# Autodesk Inventor assembly: SingleOmniWheelAssembly
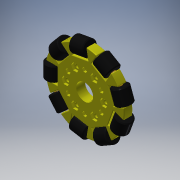
[picture p0: Inventor's stored thumbnail of the model, 180x180]
Saved by Autodesk Inventor 2016 (Build 200138000, 138)
## iProperties
Created: 2016-12-01
Part Number: SingleOmniWheelAssembly
Document SubType Name: Assembly
Designer: Evan Phil George
Author: Evan Phil George
## Documents named in this file (3)
- C:\Users\Evan Phil George\Desktop\Ball Balancing Robot\TestBenchInventor\OmniWheel\SingleOmniWheelAssembly.iam
- C:\Users\Evan Phil George\Desktop\Ball Balancing Robot\TestBenchInventor\OmniWheel\Frame.ipt
- C:\Users\Evan Phil George\Desktop\Ball Balancing Robot\TestBenchInventor\OmniWheel\RollerAxleWasherSubAssembly.iam
## Components (11 placed, 2 different names)
1. Frame:1 — Mate:1, Mate:2, Mate:3, Mate:4, Mate:5, Mate:6, Mate:7, Mate:8, Mate:9, Mate:10, Mate:11, Mate:12, Mate:13, Mate:14, Mate:15, Mate:16, Mate:17, Mate:18, Mate:19, Mate:20, Mate:21
2. RollerAxleWasherSubAssembly:1 [sub-assembly] — Mate:1, Mate:2
3. RollerAxleWasherSubAssembly:2 [sub-assembly] — Mate:3, Mate:4
4. RollerAxleWasherSubAssembly:3 [sub-assembly] — Mate:5, Mate:6
5. RollerAxleWasherSubAssembly:4 [sub-assembly] — Mate:7, Mate:8
6. RollerAxleWasherSubAssembly:5 [sub-assembly] — Mate:9, Mate:10
7. RollerAxleWasherSubAssembly:6 [sub-assembly] — Mate:11, Mate:12
8. RollerAxleWasherSubAssembly:7 [sub-assembly] — Mate:13, Mate:14
9. RollerAxleWasherSubAssembly:8 [sub-assembly] — Mate:15, Mate:16
10. RollerAxleWasherSubAssembly:9 [sub-assembly] — Mate:17, Mate:18
11. Frame:2 — Mate:19, Mate:20, Mate:21
## Relationships (21: Mate 21)
- Mate:1: Frame:1 ↔ RollerAxleWasherSubAssembly:1
- Mate:2 (0.5 mm): Frame:1 ↔ RollerAxleWasherSubAssembly:1
- Mate:3: Frame:1 ↔ RollerAxleWasherSubAssembly:2
- Mate:4 (0.5 mm): Frame:1 ↔ RollerAxleWasherSubAssembly:2
- Mate:5: Frame:1 ↔ RollerAxleWasherSubAssembly:3
- Mate:6 (0.5 mm): Frame:1 ↔ RollerAxleWasherSubAssembly:3
- Mate:7: Frame:1 ↔ RollerAxleWasherSubAssembly:4
- Mate:8 (0.5 mm): Frame:1 ↔ RollerAxleWasherSubAssembly:4
- Mate:9: Frame:1 ↔ RollerAxleWasherSubAssembly:5
- Mate:10 (0.5 mm): Frame:1 ↔ RollerAxleWasherSubAssembly:5
- Mate:11: Frame:1 ↔ RollerAxleWasherSubAssembly:6
- Mate:12 (0.5 mm): Frame:1 ↔ RollerAxleWasherSubAssembly:6
- Mate:13: Frame:1 ↔ RollerAxleWasherSubAssembly:7
- Mate:14 (0.5 mm): Frame:1 ↔ RollerAxleWasherSubAssembly:7
- Mate:15: Frame:1 ↔ RollerAxleWasherSubAssembly:8
- Mate:16 (0.5 mm): Frame:1 ↔ RollerAxleWasherSubAssembly:8
- Mate:17: Frame:1 ↔ RollerAxleWasherSubAssembly:9
- Mate:18 (0.5 mm): Frame:1 ↔ RollerAxleWasherSubAssembly:9
- Mate:19: Frame:1 ↔ Frame:2
- Mate:20: Frame:1 ↔ Frame:2
- Mate:21: Frame:1 ↔ Frame:2
